# Autodesk Inventor assembly: Rover
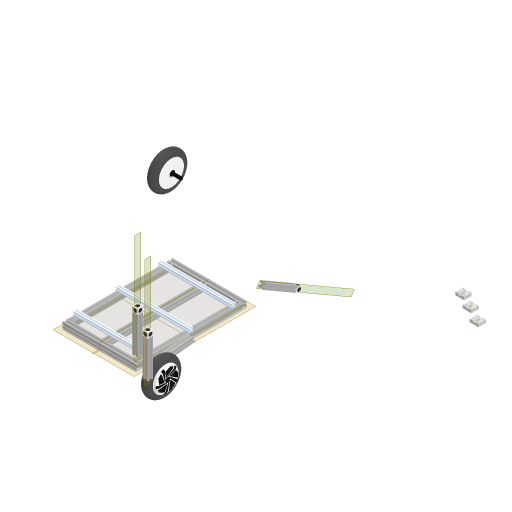
[picture p0: Inventor's stored thumbnail of the model, 512x512]
Saved by Autodesk Inventor 2023.2 (Build 272271030, 271C)
## iProperties
Created: 2024-10-30
Part Number: Rover
Document SubType Name: Assembly
Designer: I9232
Author: I9232
## Documents named in this file (8)
- D:\!Cheburashka\Cheburashka_construction\Rover\Rover.iam
- D:\!Cheburashka\Cheburashka_construction\Rover\platform.ipt
- D:\!Cheburashka\Cheburashka_construction\Rover\Motor, BLDC, Hoverboard Wheel, 8.0in.ipt
- D:\!Cheburashka\Cheburashka_construction\Rover\Деталь14.ipt
- D:\!Cheburashka\Cheburashka_construction\Rover\SHF16\SHF16.ipt
- D:\!Cheburashka\Cheburashka_construction\Rover\Profil 20x20.ipt
- D:\!Cheburashka\Cheburashka_construction\Rover\snsd.30.52.93._3_kh_storonniy_kubicheskiy_soedinitel_30kh30_d_paz_8_s165_\snsd.30.52.93._3_kh_storonniy_kubicheskiy_soedinitel_30kh30_d_paz_8_s165_.iam
- D:\!Cheburashka\Cheburashka_construction\Rover\Крепление мотора.ipt
## Components (31 placed, 7 different names)
1. platform:1 — Совмещение:1, Совмещение:2, Совмещение:3, Совмещение:4, Совмещение:14, Совмещение:15, Совмещение:27, Совмещение:54, Совмещение:55, Совмещение:56, Совмещение:57, Совмещение:58, Совмещение:59, Совмещение:61, Совмещение:62
2. Motor, BLDC, Hoverboard Wheel, 8.0in:3 — Совмещение:85, Совмещение:86
3. Motor, BLDC, Hoverboard Wheel, 8.0in:4
4. Motor, BLDC, Hoverboard Wheel, 8.0in:5
5. Motor, BLDC, Hoverboard Wheel, 8.0in:6
6. профиль 30x30:3 — Совмещение:3, Совмещение:15, Совмещение:20, Совмещение:21, Совмещение:22, Совмещение:23, Совмещение:24, Совмещение:25, Совмещение:76, Совмещение:77
7. профиль 30x30:4 — Совмещение:4, Совмещение:14, Совмещение:60
8. SHF16:1 — Совмещение:53
9. SHF16:2
10. SHF16:3 — Совмещение:47
11. SHF16:4 — Совмещение:48
12. SHF16:5 — Совмещение:49
13. SHF16:6 — Совмещение:51
14. Profil 20x20:1 — Совмещение:24, Совмещение:25, Совмещение:53
15. Profil 20x20:2 — Совмещение:20, Совмещение:21, Совмещение:27, Совмещение:28, Совмещение:47, Совмещение:49
16. Profil 20x20:3 — Совмещение:22, Совмещение:23, Совмещение:28, Совмещение:48, Совмещение:51
17. профиль 30x30:5 — Совмещение:55, Совмещение:58, Совмещение:59, Совмещение:63
18. профиль 30x30:6 — Совмещение:54, Совмещение:56, Совмещение:57, Совмещение:60
19. профиль 30x30:7 — Совмещение:61, Совмещение:62, Совмещение:63
20. профиль 30x30:8 — Совмещение:69, Совмещение:70, Совмещение:75
21. профиль 30x30:9 — Совмещение:71, Совмещение:72, Совмещение:74
22. профиль 30x30:10 — Совмещение:67, Совмещение:68, Совмещение:73, Совмещение:76
23. профиль 30x30:11 — Совмещение:64, Совмещение:65, Совмещение:66, Совмещение:77
24. snsd.30.52.93._3_kh_storonniy_kubicheskiy_soedinitel_30kh30_d_paz_8_s165_:1 [sub-assembly] — Совмещение:64, Совмещение:65, Совмещение:66
25. snsd.30.52.93._3_kh_storonniy_kubicheskiy_soedinitel_30kh30_d_paz_8_s165_:2 [sub-assembly] — Совмещение:67, Совмещение:68, Совмещение:73, Совмещение:78, Совмещение:82, Совмещение:83
26. snsd.30.52.93._3_kh_storonniy_kubicheskiy_soedinitel_30kh30_d_paz_8_s165_:3 [sub-assembly] — Совмещение:71, Совмещение:72, Совмещение:74
27. snsd.30.52.93._3_kh_storonniy_kubicheskiy_soedinitel_30kh30_d_paz_8_s165_:4 [sub-assembly] — Совмещение:69, Совмещение:70, Совмещение:75
28. Нижняя часть крепления мотора:1 — Совмещение:78, Совмещение:82, Совмещение:83, Совмещение:85, Совмещение:86
29. Нижняя часть крепления мотора:2
30. Нижняя часть крепления мотора:3
31. Нижняя часть крепления мотора:4
## Relationships (48: Mate 48)
- Совмещение:1 [Mate]: platform:1
- Совмещение:2 [Mate]: platform:1
- Совмещение:3 [Mate]: platform:1 ↔ профиль 30x30:3
- Совмещение:4 [Mate]: platform:1 ↔ профиль 30x30:4
- Совмещение:14 [Mate]: platform:1 ↔ профиль 30x30:4
- Совмещение:15 [Mate]: platform:1 ↔ профиль 30x30:3
- Совмещение:20 [Mate]: профиль 30x30:3 ↔ Profil 20x20:2
- Совмещение:21 [Mate]: профиль 30x30:3 ↔ Profil 20x20:2
- Совмещение:22 [Mate]: профиль 30x30:3 ↔ Profil 20x20:3
- Совмещение:23 [Mate]: профиль 30x30:3 ↔ Profil 20x20:3
- Совмещение:24 [Mate]: профиль 30x30:3 ↔ Profil 20x20:1
- Совмещение:25 [Mate]: профиль 30x30:3 ↔ Profil 20x20:1
- Совмещение:27 [Mate] (60 mm): platform:1 ↔ Profil 20x20:2
- Совмещение:28 [Mate] (210 mm): Profil 20x20:2 ↔ Profil 20x20:3
- Совмещение:47 [Mate]: SHF16:3 ↔ Profil 20x20:2
- Совмещение:48 [Mate]: SHF16:4 ↔ Profil 20x20:3
- Совмещение:49 [Mate]: SHF16:5 ↔ Profil 20x20:2
- Совмещение:51 [Mate]: SHF16:6 ↔ Profil 20x20:3
- Совмещение:53 [Mate]: SHF16:1 ↔ Profil 20x20:1
- Совмещение:54 [Mate]: platform:1 ↔ профиль 30x30:6
- Совмещение:55 [Mate]: platform:1 ↔ профиль 30x30:5
- Совмещение:56 [Mate]: platform:1 ↔ профиль 30x30:6
- Совмещение:57 [Mate]: platform:1 ↔ профиль 30x30:6
- Совмещение:58 [Mate]: platform:1 ↔ профиль 30x30:5
- Совмещение:59 [Mate]: platform:1 ↔ профиль 30x30:5
- Совмещение:60 [Mate]: профиль 30x30:4 ↔ профиль 30x30:6
- Совмещение:61 [Mate]: platform:1 ↔ профиль 30x30:7
- Совмещение:62 [Mate]: platform:1 ↔ профиль 30x30:7
- Совмещение:63 [Mate]: профиль 30x30:5 ↔ профиль 30x30:7
- Совмещение:64 [Mate]: профиль 30x30:11 ↔ snsd.30.52.93._3_kh_storonniy_kubicheskiy_soedinitel_30kh30_d_paz_8_s165_:1
- Совмещение:65 [Mate]: профиль 30x30:11 ↔ snsd.30.52.93._3_kh_storonniy_kubicheskiy_soedinitel_30kh30_d_paz_8_s165_:1
- Совмещение:66 [Mate]: профиль 30x30:11 ↔ snsd.30.52.93._3_kh_storonniy_kubicheskiy_soedinitel_30kh30_d_paz_8_s165_:1
- Совмещение:67 [Mate]: профиль 30x30:10 ↔ snsd.30.52.93._3_kh_storonniy_kubicheskiy_soedinitel_30kh30_d_paz_8_s165_:2
- Совмещение:68 [Mate]: профиль 30x30:10 ↔ snsd.30.52.93._3_kh_storonniy_kubicheskiy_soedinitel_30kh30_d_paz_8_s165_:2
- Совмещение:69 [Mate]: профиль 30x30:8 ↔ snsd.30.52.93._3_kh_storonniy_kubicheskiy_soedinitel_30kh30_d_paz_8_s165_:4
- Совмещение:70 [Mate]: профиль 30x30:8 ↔ snsd.30.52.93._3_kh_storonniy_kubicheskiy_soedinitel_30kh30_d_paz_8_s165_:4
- Совмещение:71 [Mate]: профиль 30x30:9 ↔ snsd.30.52.93._3_kh_storonniy_kubicheskiy_soedinitel_30kh30_d_paz_8_s165_:3
- Совмещение:72 [Mate]: профиль 30x30:9 ↔ snsd.30.52.93._3_kh_storonniy_kubicheskiy_soedinitel_30kh30_d_paz_8_s165_:3
- Совмещение:73 [Mate]: профиль 30x30:10 ↔ snsd.30.52.93._3_kh_storonniy_kubicheskiy_soedinitel_30kh30_d_paz_8_s165_:2
- Совмещение:74 [Mate]: профиль 30x30:9 ↔ snsd.30.52.93._3_kh_storonniy_kubicheskiy_soedinitel_30kh30_d_paz_8_s165_:3
- Совмещение:75 [Mate]: профиль 30x30:8 ↔ snsd.30.52.93._3_kh_storonniy_kubicheskiy_soedinitel_30kh30_d_paz_8_s165_:4
- Совмещение:76 [Mate]: профиль 30x30:3 ↔ профиль 30x30:10
- Совмещение:77 [Mate]: профиль 30x30:3 ↔ профиль 30x30:11
- Совмещение:78 [Mate]: snsd.30.52.93._3_kh_storonniy_kubicheskiy_soedinitel_30kh30_d_paz_8_s165_:2 ↔ Нижняя часть крепления мотора:1
- Совмещение:82 [Mate]: snsd.30.52.93._3_kh_storonniy_kubicheskiy_soedinitel_30kh30_d_paz_8_s165_:2 ↔ Нижняя часть крепления мотора:1
- Совмещение:83 [Mate]: snsd.30.52.93._3_kh_storonniy_kubicheskiy_soedinitel_30kh30_d_paz_8_s165_:2 ↔ Нижняя часть крепления мотора:1
- Совмещение:85 [Mate]: Motor, BLDC, Hoverboard Wheel, 8.0in:3 ↔ Нижняя часть крепления мотора:1
- Совмещение:86 [Mate]: Motor, BLDC, Hoverboard Wheel, 8.0in:3 ↔ Нижняя часть крепления мотора:1
